# Autodesk Inventor assembly: Incubator
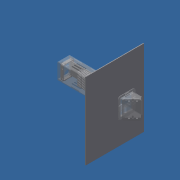
[picture p0: Inventor's stored thumbnail of the model, 180x180]
Saved by Autodesk Inventor 2016 (Build 200138000, 138)
## iProperties
Created: 2016-04-03
Part Number: Incubator
Document SubType Name: Assembly
Designer: admin
Author: admin
## Documents named in this file (15)
- E:\Alex\Incubator\Incubator.iam
- E:\Alex\Incubator\Wall.ipt
- E:\Alex\Incubator\Top.ipt
- E:\Alex\Incubator\Front_panel.ipt
- E:\Alex\Incubator\Bottom.ipt
- E:\Alex\Incubator\Fan_plate.ipt
- E:\Alex\Incubator\Fan.ipt
- E:\Alex\Incubator\Heat_sink.ipt
- E:\Alex\Incubator\Heater_pcb.ipt
- E:\Alex\Incubator\Front_stopper.ipt
- E:\Alex\Incubator\Front_stopper2.ipt
- E:\Alex\Incubator\Cardboard_front.ipt
- E:\Alex\Incubator\Pin.ipt
- E:\Alex\Incubator\Back_plate.ipt
- E:\Alex\Incubator\Board_holder.ipt
## Components (18 placed, 14 different names)
1. Wall:1 — Flush:2, Tangent:2, Mate:4, Mate:6, Mate:9, Mate:10, Mate:32, Mate:38, Mate:43, Mate:47
2. Wall:2 — Flush:5, Mate:3, Tangent:1, Tangent:3, Mate:5, Mate:7, Mate:8, Mate:13, Mate:35, Mate:46, Mate:55
3. Top:1 — Flush:2, Flush:5, Mate:4, Mate:5, Mate:6, Mate:7, Mate:27, Mate:28, Mate:31, Mate:34, Mate:36, Mate:39, Mate:40, Mate:45
4. Front_panel:1 — Mate:3, Tangent:1, Tangent:2, Tangent:3
5. Bottom:1 — Mate:8, Mate:9, Mate:10, Mate:44, Mate:48, Mate:49, Mate:54, Mate:56, Mate:57
6. Fan_plate:1 — Mate:13, Mate:14, Mate:15, Mate:16, Mate:44, Mate:46
7. Fan:1 — Mate:14, Mate:15, Mate:16
8. Heat_sink:1 — Mate:17, Flush:6, Flush:7
9. Heater_pcb:1 — Mate:17, Flush:6, Flush:7, Mate:43, Mate:50, Mate:51, Flush:9, Mate:52, Flush:10, Mate:53
10. Front_stopper:1 — Mate:27, Mate:28, Mate:30, Mate:57
11. Front_stopper2:1 — Mate:30, Mate:31, Mate:32, Mate:33
12. Cardboard_front:1 — Mate:33, Mate:34, Mate:35, Mate:37
13. Front_stopper2:2 — Mate:36, Mate:37, Mate:38, Mate:41, Mate:42
14. Pin:1 — Mate:39, Flush:8, Mate:42
15. Pin:2 — Mate:40, Flush:8, Mate:41, Mate:45
16. Back_plate:1 — Mate:47, Mate:48, Mate:49
17. Board_holder:1 — Mate:50, Flush:10, Mate:53, Mate:54, Mate:55
18. Board_holder:2 — Mate:51, Flush:9, Mate:52, Mate:56
## Relationships (53: Mate 43, Flush 7, Tangent 3)
- Flush:2: Wall:1 ↔ Top:1
- Flush:5: Wall:2 ↔ Top:1
- Mate:3: Wall:2 ↔ Front_panel:1
- Tangent:1: Wall:2 ↔ Front_panel:1
- Tangent:2: Wall:1 ↔ Front_panel:1
- Tangent:3: Wall:2 ↔ Front_panel:1
- Mate:4: Wall:1 ↔ Top:1
- Mate:5: Wall:2 ↔ Top:1
- Mate:6: Wall:1 ↔ Top:1
- Mate:7: Wall:2 ↔ Top:1
- Mate:8: Wall:2 ↔ Bottom:1
- Mate:9: Wall:1 ↔ Bottom:1
- Mate:10: Wall:1 ↔ Bottom:1
- Mate:13: Wall:2 ↔ Fan_plate:1
- Mate:14: Fan_plate:1 ↔ Fan:1
- Mate:15: Fan_plate:1 ↔ Fan:1
- Mate:16: Fan_plate:1 ↔ Fan:1
- Mate:17 (5 mm): Heat_sink:1 ↔ Heater_pcb:1
- Flush:6: Heat_sink:1 ↔ Heater_pcb:1
- Flush:7 (10 mm): Heat_sink:1 ↔ Heater_pcb:1
- Mate:27: Top:1 ↔ Front_stopper:1
- Mate:28: Top:1 ↔ Front_stopper:1
- Mate:30: Front_stopper:1 ↔ Front_stopper2:1
- Mate:31: Top:1 ↔ Front_stopper2:1
- Mate:32: Wall:1 ↔ Front_stopper2:1
- Mate:33: Front_stopper2:1 ↔ Cardboard_front:1
- Mate:34: Top:1 ↔ Cardboard_front:1
- Mate:35: Wall:2 ↔ Cardboard_front:1
- Mate:36: Top:1 ↔ Front_stopper2:2
- Mate:37: Cardboard_front:1 ↔ Front_stopper2:2
- Mate:38: Wall:1 ↔ Front_stopper2:2
- Mate:39: Top:1 ↔ Pin:1
- Mate:40: Top:1 ↔ Pin:2
- Flush:8: Pin:1 ↔ Pin:2
- Mate:41: Front_stopper2:2 ↔ Pin:2
- Mate:42: Front_stopper2:2 ↔ Pin:1
- Mate:43 (3 mm): Wall:1 ↔ Heater_pcb:1
- Mate:44: Bottom:1 ↔ Fan_plate:1
- Mate:45: Top:1 ↔ Pin:2
- Mate:46: Wall:2 ↔ Fan_plate:1
- Mate:47: Wall:1 ↔ Back_plate:1
- Mate:48: Bottom:1 ↔ Back_plate:1
- Mate:49: Bottom:1 ↔ Back_plate:1
- Mate:50: Heater_pcb:1 ↔ Board_holder:1
- Mate:51: Heater_pcb:1 ↔ Board_holder:2
- Flush:9 (-5 mm): Heater_pcb:1 ↔ Board_holder:2
- Mate:52: Heater_pcb:1 ↔ Board_holder:2
- Flush:10 (-5 mm): Heater_pcb:1 ↔ Board_holder:1
- Mate:53: Heater_pcb:1 ↔ Board_holder:1
- Mate:54: Bottom:1 ↔ Board_holder:1
- Mate:55: Wall:2 ↔ Board_holder:1
- Mate:56: Bottom:1 ↔ Board_holder:2
- Mate:57: Bottom:1 ↔ Front_stopper:1
